# Autodesk Inventor assembly: MetalCableBraider
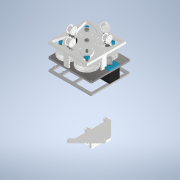
[picture p0: Inventor's stored thumbnail of the model, 180x180]
Saved by Autodesk Inventor 2022 (Build 260153000, 153)
## iProperties
Created: 2020-07-21
Part Number: MetalCableBraider
Document SubType Name: Assembly
Designer: elmar
Author: elmar
## Documents named in this file (14)
- C:\repo\FourWireBraidingMachine\InventorFiles\MetalCableBraider.iam
- C:\repo\FourWireBraidingMachine\InventorFiles\WinderAssembly.iam
- C:\repo\FourWireBraidingMachine\InventorFiles\Carriage.iam
- C:\repo\FourWireBraidingMachine\InventorFiles\NEMA17.ipt
- C:\repo\FourWireBraidingMachine\InventorFiles\ElectronicsPlate.ipt
- C:\repo\FourWireBraidingMachine\InventorFiles\GuidePlateV1.ipt
- C:\repo\FourWireBraidingMachine\InventorFiles\DriveGearNEMA17.ipt
- C:\repo\FourWireBraidingMachine\InventorFiles\BasePlateMetal.ipt
- C:\repo\FourWireBraidingMachine\InventorFiles\TwoPartHornGear.ipt
- C:\Users\Eric\OneDrive\Documents\Inventor\Content Center Files\R2022\en-US\DIN 934\DIN 934 - M8 x 1.25.ipt
- C:\Users\Eric\OneDrive\Documents\Inventor\Content Center Files\R2022\en-US\BS 4320(4)\BS 4320 - M8 (Form C).ipt
- C:\Users\Eric\OneDrive\Documents\Inventor\Content Center Files\R2022\en-US\GB_T 276-94\Rolling bearing 608 GB_T 276-94.ipt
- C:\repo\FourWireBraidingMachine\InventorFiles\Standoff.ipt
- C:\repo\FourWireBraidingMachine\InventorFiles\DIN 7991 - M8x65 Fully Threaded.ipt
## Components (31 placed, 13 different names)
1. BasePlateMetal:1 — Insert:61, Insert:64, Insert:70, Mate:2, Insert:71, Mate:3, Flush:2, Flush:3, Insert:72, Insert:74, Insert:75
2. GuidePlateV1:1 — Insert:59, Insert:60, Insert:62, Insert:63, Flush:2, Flush:3, Insert:73, Angle:2, Mate:6, Mate:8, Mate:9, Mate:10
3. WinderAssembly:1 [sub-assembly]
4. Carriage:1 [sub-assembly] — Mate:9
5. NEMA17:1 — Insert:71, Mate:3, Mate:4, Angle:1
6. ElectronicsPlate:1 — Insert:70, Mate:2
7. DriveGearNEMA17:1 — Mate:4, Angle:1, Flush:1
8. DIN 934 - replaced by DIN EN 24032/28673/28674 M8:1 — Insert:59
9. DIN 934 - replaced by DIN EN 24032/28673/28674 M8:2 — Insert:60
10. DIN 934 - replaced by DIN EN 24032/28673/28674 M8:3 — Insert:61
11. DIN 934 - replaced by DIN EN 24032/28673/28674 M8:4 — Insert:62
12. DIN 934 - replaced by DIN EN 24032/28673/28674 M8:5 — Insert:63
13. DIN 934 - replaced by DIN EN 24032/28673/28674 M8:6 — Insert:64, Insert:65
14. BS 4320 Form CD M8 (Form C):1 — Insert:65, Insert:68
15. Rolling bearing GB/T 276-1994 Type 60000 and 160000 608:1 — Insert:66, Insert:68
16. DIN 7991 - M8x65 Fully Threaded:1 — Insert:74
17. Carriage:2 [sub-assembly] — Mate:10
18. Carriage:3 [sub-assembly] — Mate:6
19. Carriage:4 [sub-assembly] — Mate:8
20. Standoff:1 — Insert:72, Insert:73
21. Standoff:2
22. Standoff:3
23. Standoff:4
24. TwoPartHornGear:1 — Insert:66, Flush:1, Angle:2
25. TwoPartHornGear:2
26. TwoPartHornGear:3
27. TwoPartHornGear:4
28. DIN 7991 - M8x65 Fully Threaded:2 — Insert:75
29. DIN 7991 - M8x65 Fully Threaded:3
30. DIN 7991 - M8x65 Fully Threaded:4
31. DIN 7991 - M8x65 Fully Threaded:5
## Component patterns: (4 elements, first: Standoff:1), (4 elements, first: TwoPartHornGear:1), (4 elements, first: DIN 7991 - M8x65 Fully Threaded:2)
## Relationships (27: Insert 15, Mate 7, Flush 3, Angle 2)
- Insert:59: GuidePlateV1:1 ↔ DIN 934 - replaced by DIN EN 24032/28673/28674 M8:1
- Insert:60: GuidePlateV1:1 ↔ DIN 934 - replaced by DIN EN 24032/28673/28674 M8:2
- Insert:61: BasePlateMetal:1 ↔ DIN 934 - replaced by DIN EN 24032/28673/28674 M8:3
- Insert:62: GuidePlateV1:1 ↔ DIN 934 - replaced by DIN EN 24032/28673/28674 M8:4
- Insert:63: GuidePlateV1:1 ↔ DIN 934 - replaced by DIN EN 24032/28673/28674 M8:5
- Insert:64: BasePlateMetal:1 ↔ DIN 934 - replaced by DIN EN 24032/28673/28674 M8:6
- Insert:65: DIN 934 - replaced by DIN EN 24032/28673/28674 M8:6 ↔ BS 4320 Form CD M8 (Form C):1
- Insert:66: Rolling bearing GB/T 276-1994 Type 60000 and 160000 608:1 ↔ TwoPartHornGear:1
- Insert:68: BS 4320 Form CD M8 (Form C):1 ↔ Rolling bearing GB/T 276-1994 Type 60000 and 160000 608:1
- Insert:70 (40 mm): BasePlateMetal:1 ↔ ElectronicsPlate:1
- Mate:2: BasePlateMetal:1 ↔ ElectronicsPlate:1
- Insert:71: BasePlateMetal:1 ↔ NEMA17:1
- Mate:3: BasePlateMetal:1 ↔ NEMA17:1
- Mate:4: NEMA17:1 ↔ DriveGearNEMA17:1
- Angle:1 (180 deg): NEMA17:1 ↔ DriveGearNEMA17:1
- Flush:1: DriveGearNEMA17:1 ↔ TwoPartHornGear:1
- Flush:2: BasePlateMetal:1 ↔ GuidePlateV1:1
- Flush:3: BasePlateMetal:1 ↔ GuidePlateV1:1
- Insert:72: BasePlateMetal:1 ↔ Standoff:1
- Insert:73: GuidePlateV1:1 ↔ Standoff:1
- Insert:74: BasePlateMetal:1 ↔ DIN 7991 - M8x65 Fully Threaded:1
- Insert:75: BasePlateMetal:1 ↔ DIN 7991 - M8x65 Fully Threaded:2
- Angle:2 (0 deg): GuidePlateV1:1 ↔ TwoPartHornGear:1
- Mate:6: GuidePlateV1:1 ↔ Carriage:3
- Mate:8: GuidePlateV1:1 ↔ Carriage:4
- Mate:9: GuidePlateV1:1 ↔ Carriage:1
- Mate:10: GuidePlateV1:1 ↔ Carriage:2
